# Autodesk Inventor assembly: Assembly1
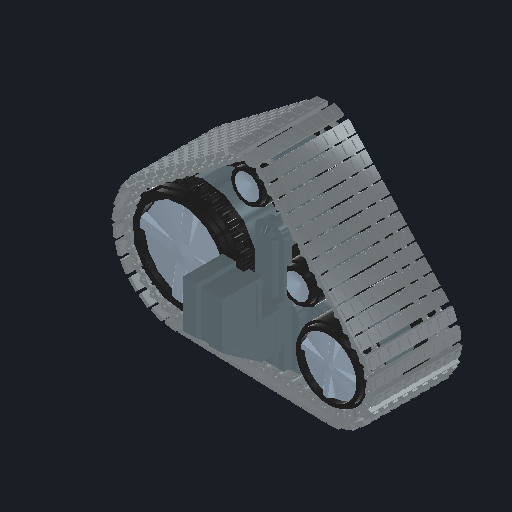
[picture p0: Inventor's stored thumbnail of the model, 512x512]
Saved by Autodesk Inventor 2022 (Build 260153000, 153)
## iProperties
Created: 2022-01-09
Part Number: Assembly1
Document SubType Name: Assembly
Designer: MatusBarany
Author: MatusBarany
## Documents named in this file (12)
- C:\Users\MatusBarany\Documents\Inventor\wall-e\matus\McCrea_pasy_zlozene_walle.iam
- C:\Users\MatusBarany\Documents\Inventor\wall-e\matus\McCrea_chrbat_walle.ipt
- C:\Users\MatusBarany\Documents\Inventor\wall-e\matus\McCrea_diel_retaze_walle.ipt
- C:\Users\MatusBarany\Documents\Inventor\wall-e\matus\McCrea_male_koleso_walle.ipt
- C:\Users\MatusBarany\Documents\Inventor\wall-e\matus\McCrea_polspojka_stredne_koleso_walle.ipt
- C:\Users\MatusBarany\Documents\Inventor\wall-e\matus\McCrea_polspojka_velke_koleso_walle.ipt
- C:\Users\MatusBarany\Documents\Inventor\wall-e\matus\McCrea_spojka_male_koleso_walle.ipt
- C:\Users\MatusBarany\Documents\Inventor\wall-e\matus\McCrea_spojka_pasy_telo_walle.ipt
- C:\Users\MatusBarany\Documents\Inventor\wall-e\matus\McCrea_stredne_koleso_walle.ipt
- C:\Users\MatusBarany\Documents\Inventor\wall-e\matus\McCrea_uchytka_walle.ipt
- C:\Users\MatusBarany\Documents\Inventor\wall-e\matus\McCrea_velke_koleso_walle.ipt
- C:\Users\Public\Documents\Autodesk\Inventor 2022\McCrea_draha_walle.ipt
## Components (68 placed, 11 different names)
1. McCrea_chrbat_walle:3 — Mate:1, Rotational:1, Mate:2, Mate:3, Mate:4, Mate:5, Mate:6
2. McCrea_male_koleso_walle:1 — Rigid:4
3. McCrea_polspojka_stredne_koleso_walle:1 — Mate:8, Flush:1, Mate:9, Rigid:2, Rigid:3
4. McCrea_polspojka_velke_koleso_walle:1 — Rigid:1, Rotational:2, Cylindrical:1, Mate:7, Mate:8, Flush:1, Mate:9
5. McCrea_spojka_male_koleso_walle:1 — Rotational:1, Rigid:4, Rigid:5, Rigid:6, Rigid:7
6. McCrea_spojka_pasy_telo_walle:1 — Mate:1, Mate:5, Mate:6
7. McCrea_velke_koleso_walle:1 — Rigid:1
8. McCrea_velke_koleso_walle:2 — Rotational:2, Flush:2
9. McCrea_stredne_koleso_walle:2 — Rigid:3
10. McCrea_uchytka_walle:1 — Mate:2, Mate:3, Mate:4, Cylindrical:1, Mate:7
11. McCrea_male_koleso_walle:2 — Rigid:7
12. McCrea_stredne_koleso_walle:3 — Rigid:2
13. McCrea_male_koleso_walle:4 — Rigid:6
14. McCrea_male_koleso_walle:5 — Rigid:5
15. McCrea_draha_walle:1 — Flush:2, Mate:10, Mate:11, Mate:12
16. McCrea_diel_retaze_walle:1 — Mate:10, Mate:11, Mate:12
17. McCrea_diel_retaze_walle:2
18. McCrea_diel_retaze_walle:3
19. McCrea_diel_retaze_walle:4
20. McCrea_diel_retaze_walle:5
21. McCrea_diel_retaze_walle:6
22. McCrea_diel_retaze_walle:7
23. McCrea_diel_retaze_walle:8
24. McCrea_diel_retaze_walle:9
25. McCrea_diel_retaze_walle:10
26. McCrea_diel_retaze_walle:11
27. McCrea_diel_retaze_walle:12
28. McCrea_diel_retaze_walle:13
29. McCrea_diel_retaze_walle:14
30. McCrea_diel_retaze_walle:15
31. McCrea_diel_retaze_walle:16
32. McCrea_diel_retaze_walle:17
33. McCrea_diel_retaze_walle:18
34. McCrea_diel_retaze_walle:19
35. McCrea_diel_retaze_walle:20
36. McCrea_diel_retaze_walle:21
37. McCrea_diel_retaze_walle:22
38. McCrea_diel_retaze_walle:23
39. McCrea_diel_retaze_walle:24
40. McCrea_diel_retaze_walle:25
41. McCrea_diel_retaze_walle:26
42. McCrea_diel_retaze_walle:27
43. McCrea_diel_retaze_walle:28
44. McCrea_diel_retaze_walle:29
45. McCrea_diel_retaze_walle:30
46. McCrea_diel_retaze_walle:31
47. McCrea_diel_retaze_walle:32
48. McCrea_diel_retaze_walle:33
49. McCrea_diel_retaze_walle:34
50. McCrea_diel_retaze_walle:35
51. McCrea_diel_retaze_walle:36
52. McCrea_diel_retaze_walle:37
53. McCrea_diel_retaze_walle:38
54. McCrea_diel_retaze_walle:39
55. McCrea_diel_retaze_walle:40
56. McCrea_diel_retaze_walle:41
57. McCrea_diel_retaze_walle:42
58. McCrea_diel_retaze_walle:43
59. McCrea_diel_retaze_walle:44
60. McCrea_diel_retaze_walle:45
61. McCrea_diel_retaze_walle:46
62. McCrea_diel_retaze_walle:47
63. McCrea_diel_retaze_walle:48
64. McCrea_diel_retaze_walle:49
65. McCrea_diel_retaze_walle:50
66. McCrea_diel_retaze_walle:51
67. McCrea_diel_retaze_walle:52
68. McCrea_diel_retaze_walle:53
## Component patterns: (53 elements, first: McCrea_diel_retaze_walle:1)
## Relationships (24: Mate 12, WeldJoint 7, RevoluteJoint 2, Flush 2, CylindricalJoint 1)
- Mate:1: McCrea_chrbat_walle:3 ↔ McCrea_spojka_pasy_telo_walle:1
- Rotational:1 [RevoluteJoint]: McCrea_chrbat_walle:3 ↔ McCrea_spojka_male_koleso_walle:1
- Rigid:1 [WeldJoint]: McCrea_polspojka_velke_koleso_walle:1 ↔ McCrea_velke_koleso_walle:1
- Rotational:2 [RevoluteJoint]: McCrea_polspojka_velke_koleso_walle:1 ↔ McCrea_velke_koleso_walle:2
- Mate:2: McCrea_chrbat_walle:3 ↔ McCrea_uchytka_walle:1
- Mate:3: McCrea_chrbat_walle:3 ↔ McCrea_uchytka_walle:1
- Mate:4: McCrea_chrbat_walle:3 ↔ McCrea_uchytka_walle:1
- Mate:5: McCrea_chrbat_walle:3 ↔ McCrea_spojka_pasy_telo_walle:1
- Mate:6: McCrea_chrbat_walle:3 ↔ McCrea_spojka_pasy_telo_walle:1
- Cylindrical:1: McCrea_polspojka_velke_koleso_walle:1 ↔ McCrea_uchytka_walle:1
- Mate:7: McCrea_polspojka_velke_koleso_walle:1 ↔ McCrea_uchytka_walle:1
- Mate:8: McCrea_polspojka_stredne_koleso_walle:1 ↔ McCrea_polspojka_velke_koleso_walle:1
- Flush:1: McCrea_polspojka_stredne_koleso_walle:1 ↔ McCrea_polspojka_velke_koleso_walle:1
- Mate:9: McCrea_polspojka_stredne_koleso_walle:1 ↔ McCrea_polspojka_velke_koleso_walle:1
- Rigid:2 [WeldJoint]: McCrea_polspojka_stredne_koleso_walle:1 ↔ McCrea_stredne_koleso_walle:3
- Rigid:3 [WeldJoint]: McCrea_polspojka_stredne_koleso_walle:1 ↔ McCrea_stredne_koleso_walle:2
- Rigid:4 [WeldJoint]: McCrea_male_koleso_walle:1 ↔ McCrea_spojka_male_koleso_walle:1
- Rigid:5 [WeldJoint]: McCrea_spojka_male_koleso_walle:1 ↔ McCrea_male_koleso_walle:5
- Rigid:6 [WeldJoint]: McCrea_spojka_male_koleso_walle:1 ↔ McCrea_male_koleso_walle:4
- Rigid:7 [WeldJoint]: McCrea_spojka_male_koleso_walle:1 ↔ McCrea_male_koleso_walle:2
- Flush:2 (-1.4986 mm): McCrea_velke_koleso_walle:2 ↔ McCrea_draha_walle:1
- Mate:10: McCrea_draha_walle:1 ↔ McCrea_diel_retaze_walle:1
- Mate:11: McCrea_draha_walle:1 ↔ McCrea_diel_retaze_walle:1
- Mate:12: McCrea_draha_walle:1 ↔ McCrea_diel_retaze_walle:1
